# Autodesk Inventor assembly: SingleBoardComputerUnit
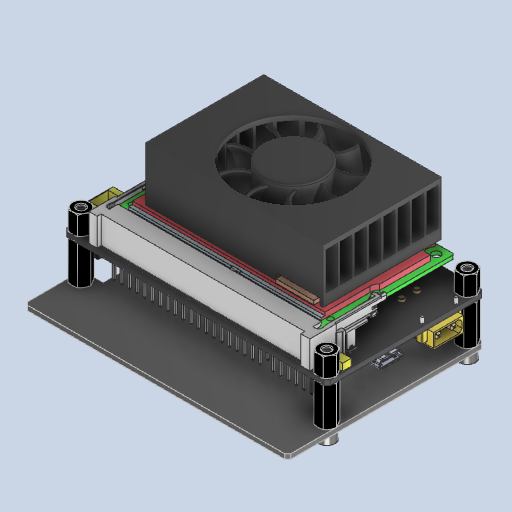
[picture p0: Inventor's stored thumbnail of the model, 512x512]
Saved by Autodesk Inventor 2022.3 (Build 263350000, 350)
## iProperties
Created: 2023-05-14
Part Number: SingleBoardComputerUnit
Document SubType Name: Assembly
Designer: Masato Kubotera
Author: Masato Kubotera
## Documents named in this file (6)
- C:\Users\Masato\Documents\Inventor\Inventor for CIT Brains\SUSTAINA-OP - Cockpit\ElectronicComponents\SingleBoardComputerUnit.iam
- C:\Users\Masato\Documents\Inventor\Inventor for CIT Brains\SUSTAINA-OP - Cockpit\ElectronicComponents\SingleBoardComputer\SingleBoardComputer.ipt
- C:\Users\Masato\Documents\Inventor\Inventor for CIT Brains\SUSTAINA-OP - Cockpit\ElectronicComponents\Board_designed_for_SUSTAINA-OP\A203-V2-Expansion-Board.ipt
- C:\Users\Masato\Documents\Inventor\Inventor for CIT Brains\SUSTAINA-OP - Cockpit\ReadyMade\Spacer\ASL-313BE.ipt
- C:\Users\Masato\Documents\Inventor\Inventor for CIT Brains\SUSTAINA-OP - Cockpit\ReadyMade\Spacer\BSL-306.5BE.ipt
- C:\Users\Masato\Documents\Inventor\Inventor for CIT Brains\SUSTAINA-OP - Cockpit\ReadyMade\Screw\UC-0306.ipt
## Components (14 placed, 5 different names)
1. SingleBoardComputer:1 — 挿入:5, 挿入:6, 挿入:7, 挿入:8, 挿入:9, 挿入:10, 挿入:11, 挿入:12
2. A203-V2-Expansion-Board:1 — フラッシュ:1, フラッシュ:2, フラッシュ:3, 挿入:1, 挿入:2, 挿入:3, 挿入:4, 挿入:13, 挿入:14, 挿入:15, 挿入:16
3. ASL-313BE:1 — 挿入:1, 挿入:5
4. ASL-313BE:2 — 挿入:2, 挿入:6
5. ASL-313BE:3 — 挿入:3, 挿入:7
6. ASL-313BE:4 — 挿入:4, 挿入:8
7. BSL-306.5BE:1 — 挿入:9
8. BSL-306.5BE:2 — 挿入:10
9. BSL-306.5BE:3 — 挿入:11
10. BSL-306.5BE:4 — 挿入:12
11. UC-0306:1 — 挿入:13
12. UC-0306:2 — 挿入:14
13. UC-0306:3 — 挿入:15
14. UC-0306:4 — 挿入:16
## Relationships (19: Insert 16, Flush 3)
- フラッシュ:1 [Flush]: A203-V2-Expansion-Board:1
- フラッシュ:2 [Flush]: A203-V2-Expansion-Board:1
- フラッシュ:3 [Flush]: A203-V2-Expansion-Board:1
- 挿入:1 [Insert]: A203-V2-Expansion-Board:1 ↔ ASL-313BE:1
- 挿入:2 [Insert]: A203-V2-Expansion-Board:1 ↔ ASL-313BE:2
- 挿入:3 [Insert]: A203-V2-Expansion-Board:1 ↔ ASL-313BE:3
- 挿入:4 [Insert]: A203-V2-Expansion-Board:1 ↔ ASL-313BE:4
- 挿入:5 [Insert]: SingleBoardComputer:1 ↔ ASL-313BE:1
- 挿入:6 [Insert]: SingleBoardComputer:1 ↔ ASL-313BE:2
- 挿入:7 [Insert]: SingleBoardComputer:1 ↔ ASL-313BE:3
- 挿入:8 [Insert]: SingleBoardComputer:1 ↔ ASL-313BE:4
- 挿入:9 [Insert]: SingleBoardComputer:1 ↔ BSL-306.5BE:1
- 挿入:10 [Insert]: SingleBoardComputer:1 ↔ BSL-306.5BE:2
- 挿入:11 [Insert]: SingleBoardComputer:1 ↔ BSL-306.5BE:3
- 挿入:12 [Insert]: SingleBoardComputer:1 ↔ BSL-306.5BE:4
- 挿入:13 [Insert]: A203-V2-Expansion-Board:1 ↔ UC-0306:1
- 挿入:14 [Insert]: A203-V2-Expansion-Board:1 ↔ UC-0306:2
- 挿入:15 [Insert]: A203-V2-Expansion-Board:1 ↔ UC-0306:3
- 挿入:16 [Insert]: A203-V2-Expansion-Board:1 ↔ UC-0306:4
